# Autodesk Inventor assembly: Shooting_BeltandBearings
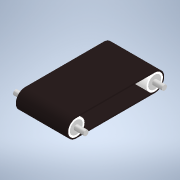
[picture p0: Inventor's stored thumbnail of the model, 180x180]
Saved by Autodesk Inventor 2020 (Build 240168000, 168)
## iProperties
Created: 2022-01-26
Part Number: Shooting_BeltandBearings
Document SubType Name: Assembly
Designer: danie
Author: danie
## Documents named in this file (6)
- C:\Users\danie\Documents\Capstone\Solidworks\Shooting_BeltandBearings.iam
- C:\Users\danie\Documents\Capstone\Solidworks\Shooting_Belt.ipt
- C:\Users\danie\Documents\Capstone\Solidworks\Shooting_Roller.ipt
- C:\Users\danie\Documents\Capstone\Solidworks\Shooting_Ball_Bearing.ipt
- C:\Users\danie\Documents\Capstone\Solidworks\1346K17_Rotary Shaft.ipt
- C:\Users\danie\Documents\Capstone\Solidworks\ShootingMech_MotorCoupling.ipt
## Components (10 placed, 5 different names)
1. Shooting_Belt:1 — Rotational:1, Rotational:2
2. Shooting_Roller:1 — Rotational:1, Rotational:3, Rotational:9
3. Shooting_Roller:2 — Rotational:2, Rotational:4, Rotational:5
4. Shooting_Ball_Bearing:1 — Rotational:3, Rotational:7
5. Shooting_Ball_Bearing:2 — Rotational:4, Rotational:6
6. Shooting_Ball_Bearing:3 — Rotational:5, Rotational:8
7. 1346K17_Rotary Shaft:1 — Rotational:6
8. 1346K17_Rotary Shaft:2 — Rotational:7
9. 1346K17_Rotary Shaft:3 — Rotational:8
10. ShootingMech_MotorCoupling:1 — Rotational:9
## Relationships (9: RevoluteJoint 9)
- Rotational:1 [RevoluteJoint]: Shooting_Belt:1 ↔ Shooting_Roller:1
- Rotational:2 [RevoluteJoint]: Shooting_Belt:1 ↔ Shooting_Roller:2
- Rotational:3 [RevoluteJoint]: Shooting_Roller:1 ↔ Shooting_Ball_Bearing:1
- Rotational:4 [RevoluteJoint]: Shooting_Roller:2 ↔ Shooting_Ball_Bearing:2
- Rotational:5 [RevoluteJoint]: Shooting_Roller:2 ↔ Shooting_Ball_Bearing:3
- Rotational:6 [RevoluteJoint]: Shooting_Ball_Bearing:2 ↔ 1346K17_Rotary Shaft:1
- Rotational:7 [RevoluteJoint]: Shooting_Ball_Bearing:1 ↔ 1346K17_Rotary Shaft:2
- Rotational:8 [RevoluteJoint]: Shooting_Ball_Bearing:3 ↔ 1346K17_Rotary Shaft:3
- Rotational:9 [RevoluteJoint] (6.35 mm): Shooting_Roller:1 ↔ ShootingMech_MotorCoupling:1
